# Autodesk Inventor assembly: daisen_motor
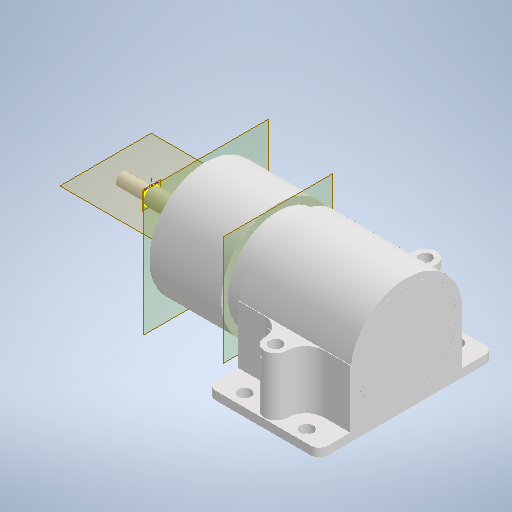
[picture p0: Inventor's stored thumbnail of the model, 512x512]
Saved by Autodesk Inventor 2025.2 (Build 292293000, 293)
## iProperties
Created: 2025-01-13
Part Number: daisen_motor
Document SubType Name: Assembly
Designer: mahhy
Author: mahhy
## Documents named in this file (4)
- D:\兵庫県立大\creap\daisen_motor.iam
- D:\兵庫県立大\creap\daisen_moto_parts1.ipt
- D:\兵庫県立大\creap\daisen_moto_parts2.ipt
- D:\兵庫県立大\creap\daisen_motor.ipt
## Components (3 placed, 3 different names)
1. daisen_moto_parts1:1 — リジッド:1
2. daisen_moto_parts2:1 — リジッド:1, 挿入:1
3. daisen_motor:1 — 挿入:1
## Relationships (2: WeldJoint 1, Insert 1)
- リジッド:1 [WeldJoint]: daisen_moto_parts1:1 ↔ daisen_moto_parts2:1
- 挿入:1 [Insert]: daisen_moto_parts2:1 ↔ daisen_motor:1
